# Autodesk Inventor assembly: LS1-100
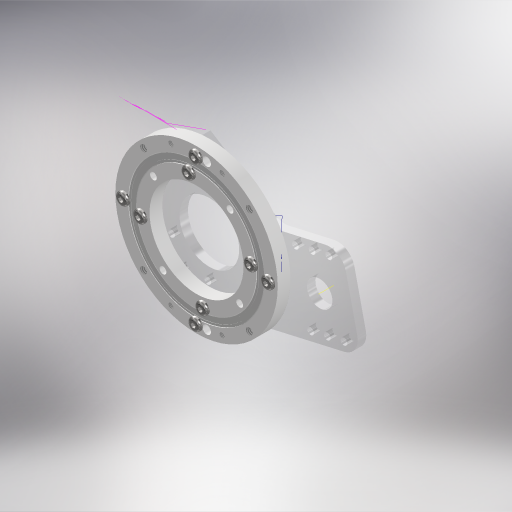
[picture p0: Inventor's stored thumbnail of the model, 512x512]
Saved by Autodesk Inventor 2023.4 (Build 274418000, 418)
## iProperties
Created: 2025-03-08
Part Number: LS1-100
Document SubType Name: Assembly
Designer: jmcintyr
Author: jmcintyr
## Documents named in this file (7)
- C:\Users\jmcintyr\Desktop\2025-ReefScape---CAD\COMMON PARTS\Lazy Suzan\LS1-100.iam
- C:\Users\jmcintyr\Desktop\2025-ReefScape---CAD\COMMON PARTS\Lazy Suzan\LS-001.ipt
- C:\Users\jmcintyr\Desktop\2025-ReefScape---CAD\COMMON PARTS\Lazy Suzan\Bearing.ipt
- C:\Users\jmcintyr\Desktop\2025-ReefScape---CAD\COMMON PARTS\Lazy Suzan\LS-002.ipt
- C:\Users\jmcintyr\Desktop\2025-ReefScape---CAD\COMMON PARTS\Lazy Suzan\2m 64t herringbone.ipt
- C:\Users\jmcintyr\Documents\Inventor\Content Center Files\R2023\en-US\ANSI B18.3(03)\ANSI B18.3 - 10-32 UNF - UNF - 0.25(1).ipt
- C:\Users\jmcintyr\Desktop\2025-ReefScape---CAD\COMMON PARTS\Lazy Suzan\GP6-004.ipt
## Components (13 placed, 6 different names)
1. LS-001:1 — Insert:1, Insert:9, Insert:10, Insert:11, Insert:12, Mate:1
2. Bearing:1 — Insert:1, Insert:8, Insert:21
3. LS-002:1 — Insert:8, Insert:13, Insert:14, Insert:15, Insert:16, Insert:17, Insert:20
4. 2m 64t herringbone:1 — Mate:1, Insert:17, Insert:21
5. Hexagon Socket Button Head Cap Screw - Inch No. 10-32 - 1/4:1 — Insert:9
6. Hexagon Socket Button Head Cap Screw - Inch No. 10-32 - 1/4:2 — Insert:10
7. Hexagon Socket Button Head Cap Screw - Inch No. 10-32 - 1/4:3 — Insert:11
8. Hexagon Socket Button Head Cap Screw - Inch No. 10-32 - 1/4:4 — Insert:12
9. Hexagon Socket Button Head Cap Screw - Inch No. 10-32 - 1/4:5 — Insert:13
10. Hexagon Socket Button Head Cap Screw - Inch No. 10-32 - 1/4:6 — Insert:14
11. Hexagon Socket Button Head Cap Screw - Inch No. 10-32 - 1/4:7 — Insert:16
12. Hexagon Socket Button Head Cap Screw - Inch No. 10-32 - 1/4:8 — Insert:15
13. GP6-004:1 — Insert:20
## Relationships (14: Insert 13, Mate 1)
- Insert:1: LS-001:1 ↔ Bearing:1
- Insert:8: Bearing:1 ↔ LS-002:1
- Insert:9: LS-001:1 ↔ Hexagon Socket Button Head Cap Screw - Inch No. 10-32 - 1/4:1
- Insert:10: LS-001:1 ↔ Hexagon Socket Button Head Cap Screw - Inch No. 10-32 - 1/4:2
- Insert:11: LS-001:1 ↔ Hexagon Socket Button Head Cap Screw - Inch No. 10-32 - 1/4:3
- Insert:12: LS-001:1 ↔ Hexagon Socket Button Head Cap Screw - Inch No. 10-32 - 1/4:4
- Insert:13: LS-002:1 ↔ Hexagon Socket Button Head Cap Screw - Inch No. 10-32 - 1/4:5
- Insert:14: LS-002:1 ↔ Hexagon Socket Button Head Cap Screw - Inch No. 10-32 - 1/4:6
- Insert:15: LS-002:1 ↔ Hexagon Socket Button Head Cap Screw - Inch No. 10-32 - 1/4:8
- Insert:16: LS-002:1 ↔ Hexagon Socket Button Head Cap Screw - Inch No. 10-32 - 1/4:7
- Mate:1: LS-001:1 ↔ 2m 64t herringbone:1
- Insert:17: LS-002:1 ↔ 2m 64t herringbone:1
- Insert:20: LS-002:1 ↔ GP6-004:1
- Insert:21: Bearing:1 ↔ 2m 64t herringbone:1
